# Autodesk Inventor assembly: richOnRails
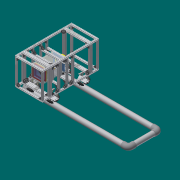
[picture p0: Inventor's stored thumbnail of the model, 180x180]
Saved by Autodesk Inventor 2016 (Build 200138000, 138)
## iProperties
Created: 2016-02-10
Part Number: richOnRails
Document SubType Name: Assembly
Designer: Sawaiz
Author: Sawaiz
## Documents named in this file (4)
- C:\Users\Sawaiz\OneDrive\projects\modularRICH\rails\richOnRails.iam
- C:\Users\Sawaiz\OneDrive\projects\modularRICH\rails\pvcRails.iam
- C:\Users\Sawaiz\OneDrive\projects\modularRICH\testMount\richWithHodoscope.iam
- C:\Users\Sawaiz\OneDrive\projects\modularRICH\rails\railFollower.iam
## Components (6 placed, 3 different names)
1. pvcRails:1 [sub-assembly]
2. richWithHodoscope:1 [sub-assembly] — Mate:1, Mate:2, Flush:3, Flush:4, Flush:5, Flush:6
3. railFollower:1 [sub-assembly] — Mate:1, Flush:4, Mate:3
4. railFollower:2 [sub-assembly] — Mate:2, Flush:1, Flush:2, Flush:3, Flush:7
5. railFollower:3 [sub-assembly] — Flush:2, Flush:5, Flush:7
6. railFollower:4 [sub-assembly] — Flush:1, Flush:6, Mate:3
## Relationships (10: Flush 7, Mate 3)
- Mate:1: richWithHodoscope:1 ↔ railFollower:1
- Mate:2: richWithHodoscope:1 ↔ railFollower:2
- Flush:1: railFollower:2 ↔ railFollower:4
- Flush:2: railFollower:2 ↔ railFollower:3
- Flush:3: richWithHodoscope:1 ↔ railFollower:2
- Flush:4: richWithHodoscope:1 ↔ railFollower:1
- Flush:5: richWithHodoscope:1 ↔ railFollower:3
- Flush:6: richWithHodoscope:1 ↔ railFollower:4
- Flush:7: railFollower:2 ↔ railFollower:3
- Mate:3: railFollower:1 ↔ railFollower:4
